# Autodesk Inventor assembly: 3.25 Traction, Circle_MIR
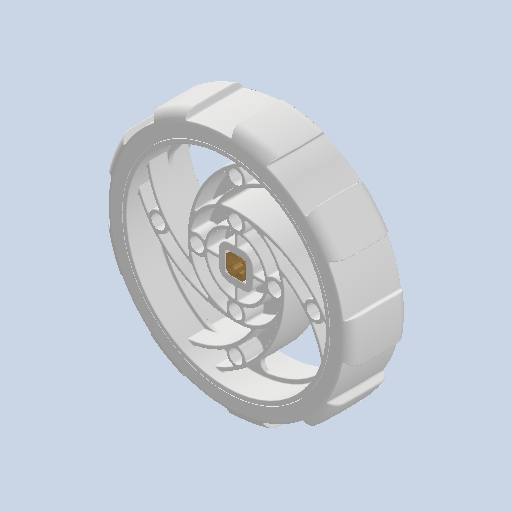
[picture p0: Inventor's stored thumbnail of the model, 512x512]
Saved by Autodesk Inventor 2024 (Build 280153000, 153)
## iProperties
Created: 2022-08-02
Part Number: 3.25 Traction, Circle_MIR
Document SubType Name: Assembly
Designer: ismae
Author: ylu12
## Documents named in this file (3)
- C:\Users\ismae\Desktop\VEX\CAD 2023\VEX-CAD-Inventor\Motion\Wheels\Traction Wheel\3.25 Traction, Circle_MIR.iam
- C:\Users\ismae\Desktop\VEX\CAD 2023\VEX-CAD-Inventor\Motion\Wheels\Reference Files\3.25 Traction_MIR.ipt
- C:\Users\ismae\Desktop\VEX\CAD 2023\VEX-CAD-Inventor\Motion\HS Shaft Adapter Circle_MIR2.ipt
## Components (2 placed, 2 different names)
1. 3.25 Traction_MIR:1 — Coincidencia:8, Coincidencia:7, Nivelación:4
2. HS Shaft Adapter Circle_MIR2:1 — Nivelación:10, Coincidencia:33, Coincidencia:32
## Relationships (6: Mate 4, Flush 2)
- Coincidencia:8 [Mate]: 3.25 Traction_MIR:1
- Coincidencia:7 [Mate]: 3.25 Traction_MIR:1
- Nivelación:4 [Flush]: 3.25 Traction_MIR:1
- Nivelación:10 [Flush] (-6.35 mm): HS Shaft Adapter Circle_MIR2:1
- Coincidencia:33 [Mate]: HS Shaft Adapter Circle_MIR2:1
- Coincidencia:32 [Mate]: HS Shaft Adapter Circle_MIR2:1
## Named parameters: Thickness = 8.255 mm
